# Autodesk Inventor assembly: !SCARA assembly
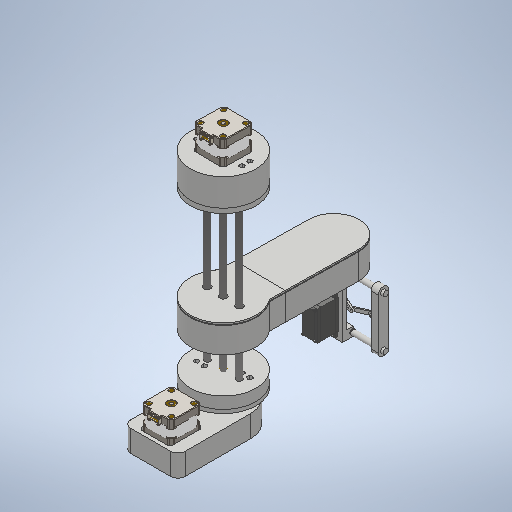
[picture p0: Inventor's stored thumbnail of the model, 512x512]
Saved by Autodesk Inventor 2025.2 (Build 292293000, 293)
## iProperties
Created: 2025-01-25
Part Number: !SCARA assembly
Document SubType Name: Assembly
Designer: caomi
Author: caomi
## Documents named in this file (21)
- C:\mnguyen\H2A\cad\SCARA\!SCARA assembly.iam
- C:\mnguyen\H2A\cad\SCARA\SCARA base.ipt
- C:\mnguyen\H2A\cad\SCARA\Stepper Motor 17HS3401.ipt
- C:\mnguyen\H2A\cad\SCARA\608 Bearing.ipt
- C:\mnguyen\H2A\cad\SCARA\Shaft support.ipt
- C:\mnguyen\H2A\cad\SCARA\SCARA swivel base - bottom.ipt
- C:\mnguyen\H2A\cad\SCARA\Guide rods.ipt
- C:\mnguyen\H2A\cad\SCARA\SCARA swivel base - mid.ipt
- C:\mnguyen\H2A\cad\SCARA\Lead screw.ipt
- C:\mnguyen\H2A\cad\SCARA\SCARA swivel connection rod.ipt
- C:\mnguyen\H2A\cad\SCARA\Bearing block.ipt
- C:\mnguyen\H2A\cad\SCARA\Lead nut.ipt
- C:\mnguyen\H2A\cad\SCARA\SCARA arm base.ipt
- C:\mnguyen\H2A\cad\SCARA\SCARA swivel top.ipt
- C:\mnguyen\H2A\cad\SCARA\Shaft coupler.ipt
- C:\mnguyen\H2A\cad\SCARA\SCARA arm.ipt
- C:\mnguyen\H2A\cad\SCARA\SCARA swivel top - lid.ipt
- C:\mnguyen\H2A\cad\SCARA\Limit_Switch.iam
- C:\mnguyen\H2A\cad\SCARA\SCARA arm base - lid.ipt
- C:\mnguyen\H2A\cad\SCARA\SCARA arm - lid.ipt
- C:\mnguyen\H2A\cad\Gripper\Gripper Assembly.iam
## Components (27 placed, 20 different names)
1. SCARA base:1 — Slider:2, Rigid:1, Swivel base bottom - SCARA base
2. Stepper Motor 17HS3401:1 — Slider:2
3. 608 Bearing:1 — Rigid:1
4. SCARA swivel base - bottom:1 — Swivel base bottom - SCARA base, Swivel base mid - bottom, Swivel connection rod - swivel base bottom
5. SCARA swivel base - mid:1 — Swivel base mid - bottom, Support block 1 - Swivel base mid, Support block 2 - Swivel base mid, Bearing - Swivel base mid
6. Shaft support:1 — Support block 2 - Swivel base mid, Smooth rod 1 - Support block 1
7. Shaft support:2 — Support block 1 - Swivel base mid, Smooth rod 2 - Support block 2
8. 608 Bearing:2 — Bearing - Swivel base mid
9. Guide rods:1 — Support block 3 - Smooth rod 1, Smooth rod 1 - Support block 1, Bearing block 1 - Smooth rod 1
10. Guide rods:2 — Support block 4 - Smooth rod 1, Smooth rod 2 - Support block 2, Bearing block 2 - Smooth rod 2
11. Lead screw:1 — Shaft coupler - Linear rod
12. SCARA swivel connection rod:1 — Swivel connection rod - swivel base bottom
13. Bearing block:1 — Bearing block 2 - Swivel arm base, Bearing block 2 - Smooth rod 2
14. Bearing block:2 — Bearing block 1 - Swivel arm base, Bearing block 1 - Smooth rod 1
15. Lead nut:1 — Lead nut - Swivel arm base
16. SCARA arm base:1 — Lead nut - Swivel arm base, Bearing block 1 - Swivel arm base, Bearing block 2 - Swivel arm base, Swivel arm - Swivel arm base, Rigid:28
17. Shaft support:3 — Support block 3 - Smooth rod 1, Swivel top - Support block 3
18. Shaft support:4 — Support block 4 - Smooth rod 1, Swivel top - Support block 4
19. SCARA swivel top:1 — Swivel top - Shaft coupler, Swivel top - Support block 3, Swivel top - Support block 4, Stepper motor - Shaft coupler, Swivel top - Swivel top lid, Limit Switch - Swivel top
20. Shaft coupler:1 — Shaft coupler - Linear rod, Swivel top - Shaft coupler
21. Stepper Motor 17HS3401:2 — Stepper motor - Shaft coupler
22. SCARA arm:1 — Swivel arm - Swivel arm base, Rigid:29, Rigid:30
23. SCARA swivel top - lid:1 — Swivel top - Swivel top lid
24. Limit_Switch:1 [sub-assembly] — Limit Switch - Swivel top
25. SCARA arm base - lid:2 — Rigid:28
26. SCARA arm - lid:1 — Rigid:29
27. Gripper Assembly:1 [sub-assembly] — Rigid:30
## Relationships (28: WeldJoint 21, RevoluteJoint 4, CylindricalJoint 2, TranslationJoint 1)
- Slider:2 [TranslationJoint]: SCARA base:1 ↔ Stepper Motor 17HS3401:1
- Rigid:1 [WeldJoint]: SCARA base:1 ↔ 608 Bearing:1
- Swivel base bottom - SCARA base [RevoluteJoint]: SCARA base:1 ↔ SCARA swivel base - bottom:1
- Swivel base mid - bottom [WeldJoint]: SCARA swivel base - bottom:1 ↔ SCARA swivel base - mid:1
- Support block 1 - Swivel base mid [WeldJoint]: SCARA swivel base - mid:1 ↔ Shaft support:2
- Support block 2 - Swivel base mid [WeldJoint]: SCARA swivel base - mid:1 ↔ Shaft support:1
- Bearing - Swivel base mid [WeldJoint]: SCARA swivel base - mid:1 ↔ 608 Bearing:2
- Swivel connection rod - swivel base bottom [WeldJoint]: SCARA swivel base - bottom:1 ↔ SCARA swivel connection rod:1
- Support block 3 - Smooth rod 1 [RevoluteJoint]: Guide rods:1 ↔ Shaft support:3
- Support block 4 - Smooth rod 1 [RevoluteJoint]: Guide rods:2 ↔ Shaft support:4
- Shaft coupler - Linear rod [WeldJoint]: Lead screw:1 ↔ Shaft coupler:1
- Swivel top - Shaft coupler [RevoluteJoint]: SCARA swivel top:1 ↔ Shaft coupler:1
- Swivel top - Support block 3 [WeldJoint]: Shaft support:3 ↔ SCARA swivel top:1
- Swivel top - Support block 4 [WeldJoint]: Shaft support:4 ↔ SCARA swivel top:1
- Stepper motor - Shaft coupler [WeldJoint]: SCARA swivel top:1 ↔ Stepper Motor 17HS3401:2
- Swivel top - Swivel top lid [WeldJoint]: SCARA swivel top:1 ↔ SCARA swivel top - lid:1
- Limit Switch - Swivel top [WeldJoint]: SCARA swivel top:1 ↔ Limit_Switch:1
- Smooth rod 1 - Support block 1 [WeldJoint]: Shaft support:1 ↔ Guide rods:1
- Smooth rod 2 - Support block 2 [WeldJoint]: Shaft support:2 ↔ Guide rods:2
- Lead nut - Swivel arm base [WeldJoint]: Lead nut:1 ↔ SCARA arm base:1
- Bearing block 1 - Swivel arm base [WeldJoint]: Bearing block:2 ↔ SCARA arm base:1
- Bearing block 2 - Swivel arm base [WeldJoint]: Bearing block:1 ↔ SCARA arm base:1
- Swivel arm - Swivel arm base [WeldJoint]: SCARA arm base:1 ↔ SCARA arm:1
- Bearing block 1 - Smooth rod 1 [CylindricalJoint]: Guide rods:1 ↔ Bearing block:2
- Bearing block 2 - Smooth rod 2 [CylindricalJoint]: Guide rods:2 ↔ Bearing block:1
- Rigid:28 [WeldJoint]: SCARA arm base:1 ↔ SCARA arm base - lid:2
- Rigid:29 [WeldJoint]: SCARA arm:1 ↔ SCARA arm - lid:1
- Rigid:30 [WeldJoint]: SCARA arm:1 ↔ Gripper Assembly:1
